# Autodesk Inventor assembly: 74. Вал первичный в сборе
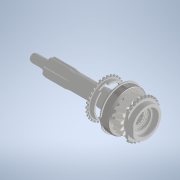
[picture p0: Inventor's stored thumbnail of the model, 180x180]
Saved by Autodesk Inventor 2021 (Build 250183000, 183)
## iProperties
Created: 2021-04-05
Part Number: 74. Вал первичный в сборе
Document SubType Name: Assembly
Designer: Данил
Author: Данил
## Documents named in this file (5)
- C:\Users\Данил\Desktop\Коробка передач\Детали\74. Вал первичный в сборе.iam
- C:\Users\Данил\Desktop\Коробка передач\Детали\74. Комплект первичного вала с кольцом после притирки.iam
- C:\Users\Данил\Desktop\Коробка передач\Детали\68. Шайба упорная.ipt
- C:\Users\Данил\Desktop\Коробка передач\Детали\68. Кольцо стопорное подшипника.ipt
- C:\Users\Данил\Desktop\Коробка передач\Детали\74. Ролик вала.ipt
## Components (17 placed, 4 different names)
1. 74. Комплект первичного вала с кольцом после притирки:1 [sub-assembly] — Совмещение:9, Касательность:1, Совмещение:14
2. 68. Шайба упорная:1 — Совмещение:12
3. 68. Кольцо стопорное подшипника:1 — Совмещение:14
4. 74. Ролик вала:1 — Совмещение:9, Совмещение:10, Касательность:1
5. 74. Ролик вала:2
6. 74. Ролик вала:3 — Совмещение:12
7. 74. Ролик вала:4
8. 74. Ролик вала:5
9. 74. Ролик вала:6
10. 74. Ролик вала:7
11. 74. Ролик вала:8
12. 74. Ролик вала:9
13. 74. Ролик вала:10
14. 74. Ролик вала:11
15. 74. Ролик вала:12
16. 74. Ролик вала:13
17. 74. Ролик вала:14
## Component patterns: (14 elements, first: 74. Ролик вала:1)
## Relationships (5: Mate 4, Tangent 1)
- Совмещение:9 [Mate]: 74. Комплект первичного вала с кольцом после притирки:1 ↔ 74. Ролик вала:1
- Совмещение:10 [Mate]: 74. Ролик вала:1
- Касательность:1 [Tangent]: 74. Комплект первичного вала с кольцом после притирки:1 ↔ 74. Ролик вала:1
- Совмещение:12 [Mate]: 68. Шайба упорная:1 ↔ 74. Ролик вала:3
- Совмещение:14 [Mate]: 74. Комплект первичного вала с кольцом после притирки:1 ↔ 68. Кольцо стопорное подшипника:1
